# Autodesk Inventor assembly: Wrist_r2
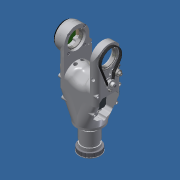
[picture p0: Inventor's stored thumbnail of the model, 180x180]
Saved by Autodesk Inventor 2016 (Build 200138000, 138)
## iProperties
Created: 2016-02-16
Part Number: Wrist_r2
Material: Generisch
Document SubType Name: Assembly
Designer: 4ndreas
Mass: 937.207 g
Surface Area: 1885 cm^2
Volume: 472.5 cm^3
Density: 1.98351 g/cm^3
Parent: R4
Author: 4ndreas
## Documents named in this file (31)
- C:\Users\4ndreas\Documents\github\Mantis-Robot-Arm\MantisRobotArm\Workspace\_Wrist_rev1\Wrist_r2.iam
- C:\Users\4ndreas\Documents\github\Mantis-Robot-Arm\MantisRobotArm\Workspace\_motors\Nema17 48.ipt
- C:\Users\4ndreas\Documents\github\Mantis-Robot-Arm\MantisRobotArm\Workspace\_Wrist_rev1\Wrist_r1\Konstruktions-Assistent\Übertragung des Zahnriemens1.iam
- C:\Users\4ndreas\Documents\github\Mantis-Robot-Arm\MantisRobotArm\Workspace\_Wrist_rev1\Wrist_r1\Konstruktions-Assistent\Übertragung des Zahnriemens2.iam
- C:\Users\4ndreas\Documents\github\Mantis-Robot-Arm\MantisRobotArm\Libraries\Content Center Files\de-DE\DIN BEARING(1)\DIN 625 SKF - SKF 61807.ipt
- C:\Users\4ndreas\Documents\github\Mantis-Robot-Arm\MantisRobotArm\Workspace\_metal parts\Synchrone Riemenscheibe16.ipt
- C:\Users\4ndreas\Documents\github\Mantis-Robot-Arm\MantisRobotArm\Workspace\_standard Parts\Distanzhuelse_M4x20mm.ipt
- C:\Users\4ndreas\Documents\github\Mantis-Robot-Arm\MantisRobotArm\Libraries\Content Center Files\de-DE\DIN 912\DIN 912 - M4 x 0,7 x 30 x 20.ipt
- C:\Users\4ndreas\Documents\github\Mantis-Robot-Arm\MantisRobotArm\Libraries\Content Center Files\de-DE\DIN 125-1  A\DIN 125 - A 4,3.ipt
- C:\Users\4ndreas\Documents\github\Mantis-Robot-Arm\MantisRobotArm\Workspace\_encoder\EncoderMagnet.ipt
- C:\Users\4ndreas\Documents\github\Mantis-Robot-Arm\MantisRobotArm\Libraries\Content Center Files\de-DE\DIN 625 - T1\DIN 625 T1 - 624 - 4 x 13 x 5.ipt
- C:\Users\4ndreas\Documents\github\Mantis-Robot-Arm\MantisRobotArm\Workspace\_metal parts\Alu_Belt_tens_3.ipt
- C:\Users\4ndreas\Documents\github\Mantis-Robot-Arm\MantisRobotArm\Workspace\_standard Parts\DIN 912 - M4 x 0,7 x50.ipt
- C:\Users\4ndreas\Documents\github\Mantis-Robot-Arm\MantisRobotArm\Libraries\Content Center Files\de-DE\DIN 912\DIN 912 - M4 x 0,7 x 16 x 14,25.ipt
- C:\Users\4ndreas\Documents\github\Mantis-Robot-Arm\MantisRobotArm\Libraries\Content Center Files\de-DE\DIN 912\DIN 912 - M3 x 0,5 x 8 x 6,75.ipt
- C:\Users\4ndreas\Documents\github\Mantis-Robot-Arm\MantisRobotArm\Libraries\Content Center Files\de-DE\DIN 125-1  A\DIN 125 - A 3,2.ipt
- C:\Users\4ndreas\Documents\github\Mantis-Robot-Arm\MantisRobotArm\Libraries\Content Center Files\de-DE\DIN 985\DIN 985 - M4.ipt
- C:\Users\4ndreas\Documents\github\Mantis-Robot-Arm\MantisRobotArm\Workspace\_Wrist_rev1\Wrist_r1\Konstruktions-Assistent\Welle1.iam
- C:\Users\4ndreas\Documents\github\Mantis-Robot-Arm\MantisRobotArm\Workspace\_Wrist_rev1\Mag4mmWelle.ipt
- C:\Users\4ndreas\Documents\github\Mantis-Robot-Arm\MantisRobotArm\Workspace\_Wrist_rev1\Wrist_EncoderMount.ipt
- C:\Users\4ndreas\Documents\github\Mantis-Robot-Arm\MantisRobotArm\Libraries\Content Center Files\de-DE\DIN 912\DIN 912 - M3 x 0,5 x 6 x 4,75.ipt
- C:\Users\4ndreas\Documents\github\Mantis-Robot-Arm\MantisRobotArm\Workspace\_encoder\encoder_neu.iam
- C:\Users\4ndreas\Documents\github\Mantis-Robot-Arm\MantisRobotArm\Workspace\_standard Parts\Slipring_SNM012A-24.ipt
- C:\Users\4ndreas\Documents\github\Mantis-Robot-Arm\MantisRobotArm\Libraries\Content Center Files\de-DE\DIN BEARING(1)\DIN 625 SKF - SKF 61802.ipt
- C:\Users\4ndreas\Documents\github\Mantis-Robot-Arm\MantisRobotArm\Workspace\_printed parts\wrist_r1_C.ipt
- C:\Users\4ndreas\Documents\github\Mantis-Robot-Arm\MantisRobotArm\Workspace\_printed parts\wrist_r1_B.ipt
- C:\Users\4ndreas\Documents\github\Mantis-Robot-Arm\MantisRobotArm\Workspace\_printed parts\wrist_r1_A.ipt
- C:\Users\4ndreas\Documents\github\Mantis-Robot-Arm\MantisRobotArm\Libraries\Content Center Files\de-DE\DIN 912\DIN 912 - M4 x 0,7 x 35 x 20.ipt
- C:\Users\4ndreas\Documents\github\Mantis-Robot-Arm\MantisRobotArm\Workspace\_printed parts\RotoatorGear_print_A.ipt
- C:\Users\4ndreas\Documents\github\Mantis-Robot-Arm\MantisRobotArm\Workspace\_printed parts\RotoatorGear_print_B.ipt
- C:\Users\4ndreas\Documents\github\Mantis-Robot-Arm\MantisRobotArm\Libraries\Content Center Files\de-DE\DIN 7991(2)\DIN 7991 - M3x16.ipt
## Components (51 placed, 29 different names)
1. wrist_r1_C:1 — Fluchtend:31, Fluchtend:32, Fluchtend:33, Passend:118, Passend:124, Passend:125, Passend:126, Passend:134, Passend:135, Passend:136, Passend:137, Passend:143, Passend:144, Passend:160
2. Nema17 48:1 — Passend:10, Passend:74, Passend:75, Passend:76, Passend:77, Passend:111, Passend:112, Passend:121, Passend:122
3. Übertragung des Zahnriemens:1 [sub-assembly] — Passend:9
4. Übertragung des Zahnriemens:2 [sub-assembly] — Passend:11, Passend:53, Passend:55, Passend:58
5. encoder_neu:1 [sub-assembly] — Passend:109, Passend:127, Passend:128
6. DIN 625 SKF SKF 61807:1 — Passend:123
7. DIN 625 SKF SKF 61807:2 — Passend:132, Passend:133
8. Synchrone Riemenscheibe1:1 — Passend:9, Passend:10, Passend:121
9. Synchrone Riemenscheibe1:2 — Passend:11, Passend:89
10. RotoatorGear_print_A:1 — Passend:145, Passend:146, Passend:147, Passend:148, Passend:150, Passend:151, Passend:152, Passend:153, Passend:159
11. DIN 912 - ersetzt durch DIN EN ISO 4762 M4 x 35:1 — Passend:141, Fluchtend:34, Fluchtend:36, Passend:144
12. DIN 912 - ersetzt durch DIN EN ISO 4762 M4 x 35:2 — Passend:142, Fluchtend:36, Passend:143
13. DIN 912 - ersetzt durch DIN EN ISO 4762 M4 x 35:3 — Passend:139, Fluchtend:35
14. DIN 912 - ersetzt durch DIN EN ISO 4762 M4 x 35:4 — Passend:140, Fluchtend:34, Fluchtend:35
15. Distanzhuelse_M4x20mm:1 — Fluchtend:37, Passend:156
16. Distanzhuelse_M4x20mm:2 — Fluchtend:37, Fluchtend:39, Passend:157
17. Distanzhuelse_M4x20mm:3 — Fluchtend:38, Fluchtend:39, Passend:154
18. Distanzhuelse_M4x20mm:4 — Passend:46, Fluchtend:38, Passend:155, Passend:158
19. DIN 912 - ersetzt durch DIN EN ISO 4762 M4 x 30:1 — Passend:142, Passend:152
20. DIN 912 - ersetzt durch DIN EN ISO 4762 M4 x 30:2 — Passend:140, Passend:151
21. DIN 912 - ersetzt durch DIN EN ISO 4762 M4 x 30:3 — Passend:139, Passend:149, Passend:150
22. DIN 912 - ersetzt durch DIN EN ISO 4762 M4 x 30:4 — Passend:46, Passend:141, Passend:153
23. EncoderMagnet:1 — Passend:101, Passend:102
24. DIN 625 - T1 624 - 4 x 13 x 5:1 — Passend:51, Passend:52, Passend:60
25. DIN 625 - T1 624 - 4 x 13 x 5:2 — Passend:51, Passend:52, Passend:53, Passend:64, Passend:65
26. Alu_Belt_tens_3:1 — Passend:55, Passend:57, Passend:59
27. DIN 125-1 A A 4,3:5 — Passend:58, Passend:59, Passend:60
28. DIN 912 - ersetzt durch DIN EN ISO 4762 M4 x 50:1 — Passend:79
29. DIN 912 - ersetzt durch DIN EN ISO 4762 M4 x 16:1 — Passend:64, Passend:65
30. DIN 912 - ersetzt durch DIN EN ISO 4762 M3 x 6:2 — Passend:66, Passend:67, Passend:74
31. DIN 125-1 A A 3,2:1 — Passend:66, Passend:67, Fluchtend:28
32. DIN 912 - ersetzt durch DIN EN ISO 4762 M3 x 8:2 — Passend:75
33. DIN 125-1 A A 3,2:2 — Fluchtend:29, Passend:112
34. DIN 912 - ersetzt durch DIN EN ISO 4762 M3 x 6:1 — Passend:77, Passend:110
35. DIN 125-1 A A 3,2:3 — Fluchtend:28, Passend:110, Passend:111
36. DIN 912 - ersetzt durch DIN EN ISO 4762 M3 x 8:4 — Passend:76
37. DIN 125-1 A A 3,2:4 — Fluchtend:29
38. DIN 985 - ersetzt durch DIN EN ISO 10511 M4:1 — Passend:79
39. Welle:1 [sub-assembly] — Passend:89
40. Mag4mmWelle:1 — Passend:101, Passend:102, Passend:115, Passend:117
41. Wrist_EncoderMount:1 — Passend:109, Passend:127, Passend:128, Passend:129, Passend:130, Passend:131
42. Slipring_SNM012A-24:1 — Passend:114, Passend:115, Passend:117, Passend:118, Passend:137
43. DIN 625 SKF SKF 61802:1 — Passend:114, Passend:146, Passend:147
44. wrist_r1_B:1 — Passend:122, Passend:123, Passend:124, Passend:125, Passend:126, Passend:129, Passend:130, Passend:131, Passend:163, Passend:164, Passend:165, Passend:166
45. wrist_r1_A:1 — Passend:132, Passend:133, Passend:134, Passend:135, Passend:136, Passend:161, Passend:162
46. RotoatorGear_print_B:1 — Passend:145, Passend:148, Passend:149, Passend:154, Passend:155, Passend:156, Passend:157, Passend:158, Passend:159, Passend:160
47. DIN 912 - ersetzt durch DIN EN ISO 4762 M4 x 30:5 — Passend:161, Passend:162
48. DIN 7991 M3x16:1 — Passend:163
49. DIN 7991 M3x16:2 — Passend:164
50. DIN 7991 M3x16:3 — Passend:165
51. DIN 7991 M3x16:4 — Passend:166
## Relationships (99: Mate 85, Flush 14)
- Passend:9 [Mate]: Übertragung des Zahnriemens:1 ↔ Synchrone Riemenscheibe1:1
- Passend:10 [Mate] (3 mm): Nema17 48:1 ↔ Synchrone Riemenscheibe1:1
- Passend:11 [Mate]: Übertragung des Zahnriemens:2 ↔ Synchrone Riemenscheibe1:2
- [Flush]: DIN 912 - ersetzt durch DIN EN ISO 4762 M4 x 30:3 ↔ DIN 912 - ersetzt durch DIN EN ISO 4762 M4 x 30:4
- [Flush]: DIN 912 - ersetzt durch DIN EN ISO 4762 M4 x 30:2 ↔ DIN 912 - ersetzt durch DIN EN ISO 4762 M4 x 30:3
- [Flush]: DIN 912 - ersetzt durch DIN EN ISO 4762 M4 x 30:1 ↔ DIN 912 - ersetzt durch DIN EN ISO 4762 M4 x 30:2
- [Mate]: Distanzhuelse_M4x20mm:3 ↔ DIN 912 - ersetzt durch DIN EN ISO 4762 M4 x 30:1
- [Mate]: Distanzhuelse_M4x20mm:2 ↔ DIN 912 - ersetzt durch DIN EN ISO 4762 M4 x 30:3
- [Mate]: Distanzhuelse_M4x20mm:1 ↔ DIN 912 - ersetzt durch DIN EN ISO 4762 M4 x 30:2
- Passend:46 [Mate]: Distanzhuelse_M4x20mm:4 ↔ DIN 912 - ersetzt durch DIN EN ISO 4762 M4 x 30:4
- Passend:51 [Mate]: DIN 625 - T1 624 - 4 x 13 x 5:1 ↔ DIN 625 - T1 624 - 4 x 13 x 5:2
- Passend:52 [Mate]: DIN 625 - T1 624 - 4 x 13 x 5:1 ↔ DIN 625 - T1 624 - 4 x 13 x 5:2
- Passend:53 [Mate]: Übertragung des Zahnriemens:2 ↔ DIN 625 - T1 624 - 4 x 13 x 5:2
- Passend:55 [Mate]: Übertragung des Zahnriemens:2 ↔ Alu_Belt_tens_3:1
- Passend:57 [Mate]: Alu_Belt_tens_3:1
- Passend:58 [Mate]: Übertragung des Zahnriemens:2 ↔ DIN 125-1 A A 4,3:5
- Passend:59 [Mate]: Alu_Belt_tens_3:1 ↔ DIN 125-1 A A 4,3:5
- Passend:60 [Mate]: DIN 625 - T1 624 - 4 x 13 x 5:1 ↔ DIN 125-1 A A 4,3:5
- Passend:64 [Mate]: DIN 625 - T1 624 - 4 x 13 x 5:2 ↔ DIN 912 - ersetzt durch DIN EN ISO 4762 M4 x 16:1
- Passend:65 [Mate]: DIN 625 - T1 624 - 4 x 13 x 5:2 ↔ DIN 912 - ersetzt durch DIN EN ISO 4762 M4 x 16:1
- Passend:66 [Mate]: DIN 912 - ersetzt durch DIN EN ISO 4762 M3 x 6:2 ↔ DIN 125-1 A A 3,2:1
- Passend:67 [Mate]: DIN 912 - ersetzt durch DIN EN ISO 4762 M3 x 6:2 ↔ DIN 125-1 A A 3,2:1
- [Mate]: DIN 912 - ersetzt durch DIN EN ISO 4762 M3 x 8:2 ↔ DIN 125-1 A A 3,2:2
- [Mate]: DIN 912 - ersetzt durch DIN EN ISO 4762 M3 x 8:2 ↔ DIN 125-1 A A 3,2:2
- [Mate]: DIN 912 - ersetzt durch DIN EN ISO 4762 M3 x 6:1 ↔ DIN 125-1 A A 3,2:3
- [Mate]: DIN 912 - ersetzt durch DIN EN ISO 4762 M3 x 8:4 ↔ DIN 125-1 A A 3,2:4
- [Mate]: DIN 912 - ersetzt durch DIN EN ISO 4762 M3 x 8:4 ↔ DIN 125-1 A A 3,2:4
- Passend:74 [Mate]: Nema17 48:1 ↔ DIN 912 - ersetzt durch DIN EN ISO 4762 M3 x 6:2
- Passend:75 [Mate]: Nema17 48:1 ↔ DIN 912 - ersetzt durch DIN EN ISO 4762 M3 x 8:2
- Passend:76 [Mate]: Nema17 48:1 ↔ DIN 912 - ersetzt durch DIN EN ISO 4762 M3 x 8:4
- Passend:77 [Mate]: Nema17 48:1 ↔ DIN 912 - ersetzt durch DIN EN ISO 4762 M3 x 6:1
- Passend:79 [Mate]: DIN 912 - ersetzt durch DIN EN ISO 4762 M4 x 50:1 ↔ DIN 985 - ersetzt durch DIN EN ISO 10511 M4:1
- Passend:89 [Mate]: Synchrone Riemenscheibe1:2 ↔ Welle:1
- Passend:101 [Mate]: EncoderMagnet:1 ↔ Mag4mmWelle:1
- Passend:102 [Mate]: EncoderMagnet:1 ↔ Mag4mmWelle:1
- Passend:109 [Mate]: encoder_neu:1 ↔ Wrist_EncoderMount:1
- Fluchtend:28 [Flush]: DIN 125-1 A A 3,2:1 ↔ DIN 125-1 A A 3,2:3
- Passend:110 [Mate]: DIN 912 - ersetzt durch DIN EN ISO 4762 M3 x 6:1 ↔ DIN 125-1 A A 3,2:3
- Passend:111 [Mate] (2 mm): Nema17 48:1 ↔ DIN 125-1 A A 3,2:3
- Fluchtend:29 [Flush]: DIN 125-1 A A 3,2:2 ↔ DIN 125-1 A A 3,2:4
- Passend:112 [Mate] (4 mm): Nema17 48:1 ↔ DIN 125-1 A A 3,2:2
- Passend:114 [Mate]: Slipring_SNM012A-24:1 ↔ DIN 625 SKF SKF 61802:1
- Passend:115 [Mate]: Mag4mmWelle:1 ↔ Slipring_SNM012A-24:1
- Passend:117 [Mate] (1 mm): Mag4mmWelle:1 ↔ Slipring_SNM012A-24:1
- Fluchtend:31 [Flush]: wrist_r1_C:1
- Fluchtend:32 [Flush]: wrist_r1_C:1
- Fluchtend:33 [Flush]: wrist_r1_C:1
- Passend:118 [Mate]: wrist_r1_C:1 ↔ Slipring_SNM012A-24:1
- Passend:121 [Mate]: Nema17 48:1 ↔ Synchrone Riemenscheibe1:1
- Passend:122 [Mate]: Nema17 48:1 ↔ wrist_r1_B:1
- Passend:123 [Mate]: DIN 625 SKF SKF 61807:1 ↔ wrist_r1_B:1
- Passend:124 [Mate]: wrist_r1_C:1 ↔ wrist_r1_B:1
- Passend:125 [Mate]: wrist_r1_C:1 ↔ wrist_r1_B:1
- Passend:126 [Mate]: wrist_r1_C:1 ↔ wrist_r1_B:1
- Passend:127 [Mate]: encoder_neu:1 ↔ Wrist_EncoderMount:1
- Passend:128 [Mate]: encoder_neu:1 ↔ Wrist_EncoderMount:1
- Passend:129 [Mate]: Wrist_EncoderMount:1 ↔ wrist_r1_B:1
- Passend:130 [Mate]: Wrist_EncoderMount:1 ↔ wrist_r1_B:1
- Passend:131 [Mate]: Wrist_EncoderMount:1 ↔ wrist_r1_B:1
- Passend:132 [Mate]: DIN 625 SKF SKF 61807:2 ↔ wrist_r1_A:1
- Passend:133 [Mate]: DIN 625 SKF SKF 61807:2 ↔ wrist_r1_A:1
- Passend:134 [Mate]: wrist_r1_C:1 ↔ wrist_r1_A:1
- Passend:135 [Mate]: wrist_r1_C:1 ↔ wrist_r1_A:1
- Passend:136 [Mate]: wrist_r1_C:1 ↔ wrist_r1_A:1
- Passend:137 [Mate] (0.5 mm): wrist_r1_C:1 ↔ Slipring_SNM012A-24:1
- Passend:139 [Mate]: DIN 912 - ersetzt durch DIN EN ISO 4762 M4 x 35:3 ↔ DIN 912 - ersetzt durch DIN EN ISO 4762 M4 x 30:3
- Passend:140 [Mate]: DIN 912 - ersetzt durch DIN EN ISO 4762 M4 x 35:4 ↔ DIN 912 - ersetzt durch DIN EN ISO 4762 M4 x 30:2
- Passend:141 [Mate]: DIN 912 - ersetzt durch DIN EN ISO 4762 M4 x 35:1 ↔ DIN 912 - ersetzt durch DIN EN ISO 4762 M4 x 30:4
- Passend:142 [Mate]: DIN 912 - ersetzt durch DIN EN ISO 4762 M4 x 35:2 ↔ DIN 912 - ersetzt durch DIN EN ISO 4762 M4 x 30:1
- Fluchtend:34 [Flush]: DIN 912 - ersetzt durch DIN EN ISO 4762 M4 x 35:1 ↔ DIN 912 - ersetzt durch DIN EN ISO 4762 M4 x 35:4
- Fluchtend:35 [Flush]: DIN 912 - ersetzt durch DIN EN ISO 4762 M4 x 35:3 ↔ DIN 912 - ersetzt durch DIN EN ISO 4762 M4 x 35:4
- Fluchtend:36 [Flush]: DIN 912 - ersetzt durch DIN EN ISO 4762 M4 x 35:1 ↔ DIN 912 - ersetzt durch DIN EN ISO 4762 M4 x 35:2
- Passend:143 [Mate]: wrist_r1_C:1 ↔ DIN 912 - ersetzt durch DIN EN ISO 4762 M4 x 35:2
- Passend:144 [Mate]: wrist_r1_C:1 ↔ DIN 912 - ersetzt durch DIN EN ISO 4762 M4 x 35:1
- Passend:145 [Mate]: RotoatorGear_print_A:1 ↔ RotoatorGear_print_B:1
- Passend:146 [Mate]: RotoatorGear_print_A:1 ↔ DIN 625 SKF SKF 61802:1
- Passend:147 [Mate]: RotoatorGear_print_A:1 ↔ DIN 625 SKF SKF 61802:1
- Passend:148 [Mate]: RotoatorGear_print_A:1 ↔ RotoatorGear_print_B:1
- Passend:149 [Mate]: DIN 912 - ersetzt durch DIN EN ISO 4762 M4 x 30:3 ↔ RotoatorGear_print_B:1
- Passend:150 [Mate]: RotoatorGear_print_A:1 ↔ DIN 912 - ersetzt durch DIN EN ISO 4762 M4 x 30:3
- Fluchtend:37 [Flush]: Distanzhuelse_M4x20mm:1 ↔ Distanzhuelse_M4x20mm:2
- Fluchtend:38 [Flush]: Distanzhuelse_M4x20mm:3 ↔ Distanzhuelse_M4x20mm:4
- Fluchtend:39 [Flush]: Distanzhuelse_M4x20mm:2 ↔ Distanzhuelse_M4x20mm:3
- Passend:151 [Mate]: RotoatorGear_print_A:1 ↔ DIN 912 - ersetzt durch DIN EN ISO 4762 M4 x 30:2
- Passend:152 [Mate]: RotoatorGear_print_A:1 ↔ DIN 912 - ersetzt durch DIN EN ISO 4762 M4 x 30:1
- Passend:153 [Mate]: RotoatorGear_print_A:1 ↔ DIN 912 - ersetzt durch DIN EN ISO 4762 M4 x 30:4
- Passend:154 [Mate]: Distanzhuelse_M4x20mm:3 ↔ RotoatorGear_print_B:1
- Passend:155 [Mate]: Distanzhuelse_M4x20mm:4 ↔ RotoatorGear_print_B:1
- Passend:156 [Mate]: Distanzhuelse_M4x20mm:1 ↔ RotoatorGear_print_B:1
- Passend:157 [Mate]: Distanzhuelse_M4x20mm:2 ↔ RotoatorGear_print_B:1
- Passend:158 [Mate]: Distanzhuelse_M4x20mm:4 ↔ RotoatorGear_print_B:1
- Passend:159 [Mate]: RotoatorGear_print_A:1 ↔ RotoatorGear_print_B:1
- Passend:160 [Mate]: wrist_r1_C:1 ↔ RotoatorGear_print_B:1
- Passend:161 [Mate]: wrist_r1_A:1 ↔ DIN 912 - ersetzt durch DIN EN ISO 4762 M4 x 30:5
- Passend:162 [Mate]: wrist_r1_A:1 ↔ DIN 912 - ersetzt durch DIN EN ISO 4762 M4 x 30:5
- Passend:163 [Mate]: wrist_r1_B:1 ↔ DIN 7991 M3x16:1
- Passend:164 [Mate]: wrist_r1_B:1 ↔ DIN 7991 M3x16:2
- Passend:165 [Mate]: wrist_r1_B:1 ↔ DIN 7991 M3x16:3
- Passend:166 [Mate]: wrist_r1_B:1 ↔ DIN 7991 M3x16:4
## Named parameters: d82_d80 = 0 mm, d83_d81 = 0 mm, d84_d80 = 0 mm, d86_d80 = 0 mm, d87_d81 = 0 mm
